# Autodesk Inventor assembly: Logitech c270 Assembly
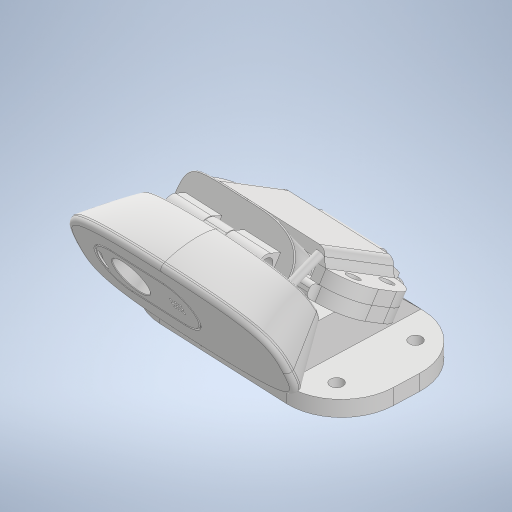
[picture p0: Inventor's stored thumbnail of the model, 512x512]
Saved by Autodesk Inventor 2023 (Build 270158000, 158)
## iProperties
Created: 2023-02-03
Part Number: Logitech c270 Assembly
Description: STEP AP203
Document SubType Name: Assembly
Designer: havie
Title: Logitech c270 Assembly.STEP
Revision Number: ANY
Sending System: SolidWorks 2021
Preprocessor: SwSTEP 2.0
## Documents named in this file (6)
- C:\Users\havie\Desktop\DO_AN_CDT\1.PART\Assembly_HCMUTE-CDT23-CAMERA_C270Logitech c270 Assembly.iam
- C:\Users\havie\Desktop\DO_AN_CDT\1.PART\Assembly_HCMUTE-CDT23-CAMERA_C270Logitech c270c.ipt
- C:\Users\havie\Desktop\DO_AN_CDT\1.PART\Assembly_HCMUTE-CDT23-CAMERA_C270Logitech c270b.ipt
- C:\Users\havie\Desktop\DO_AN_CDT\1.PART\Assembly_HCMUTE-CDT23-CAMERA_C270Logitech c270.ipt
- C:\Users\havie\Desktop\DO_AN_CDT\1.PART\Assembly_HCMUTE-CDT23-CAMERA_C270Camera Mount base.ipt
- C:\Users\havie\Desktop\DO_AN_CDT\1.PART\Assembly_HCMUTE-CDT23-CAMERA_C270attachment.ipt
## Components (5 placed, 5 different names)
1. Logitech c270c_1 — Mate:1, Mate:2, Mate:3, Mate:4, Mate:5
2. Logitech c270b_2 — Mate:4, Mate:5, Mate:9, Mate:10, Angle:1
3. Logitech c270_3 — Mate:9, Mate:10
4. Camera Mount base_4 — Mate:1, Mate:2, Mate:3, Mate:6, Mate:7, Mate:8
5. attachment_5 — Mate:6, Mate:7, Mate:8, Angle:1
## Relationships (11: Mate 10, Angle 1)
- Mate:1: Logitech c270c_1 ↔ Camera Mount base_4
- Mate:2: Logitech c270c_1 ↔ Camera Mount base_4
- Mate:3: Logitech c270c_1 ↔ Camera Mount base_4
- Mate:4: Logitech c270c_1 ↔ Logitech c270b_2
- Mate:5 (0.5 mm): Logitech c270c_1 ↔ Logitech c270b_2
- Mate:6: Camera Mount base_4 ↔ attachment_5
- Mate:7: Camera Mount base_4 ↔ attachment_5
- Mate:8: Camera Mount base_4 ↔ attachment_5
- Mate:9: Logitech c270b_2 ↔ Logitech c270_3
- Mate:10 (0.25 mm): Logitech c270b_2 ↔ Logitech c270_3
- Angle:1 (0 deg): Logitech c270b_2 ↔ attachment_5
